# Autodesk Inventor assembly: Flash_Hobby_D3536EVO
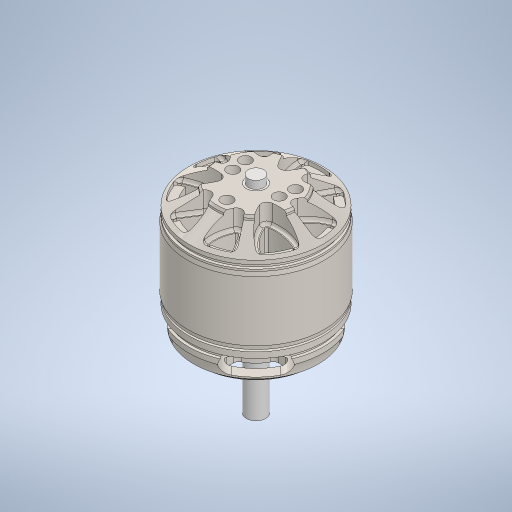
[picture p0: Inventor's stored thumbnail of the model, 512x512]
Saved by Autodesk Inventor 2023.2 (Build 272271000, 271)
## iProperties
Created: 2023-05-23
Part Number: Flash_Hobby_D3536EVO
Document SubType Name: Assembly
Designer: Nathan Cai
Mass: 105.8 g
Surface Area: 143.212 cm^2
Volume: 20.9807 cm^3
Sending System: Autodesk Translation Framework v12.4.0.73
Preprocessor: ST-DEVELOPER v19.2
Title: Flash_Hobby_D3536EVO v3.step
## Documents named in this file (4)
- E:\Documents\Inventor\Chort V2.0\Flash_Hobby_D3536EVO v3\Flash_Hobby_D3536EVO v3.iam
- E:\Documents\Inventor\Chort V2.0\Flash_Hobby_D3536EVO v3\Component1.ipt
- E:\Documents\Inventor\Chort V2.0\Flash_Hobby_D3536EVO v3\Part5.ipt
- E:\Documents\Inventor\Chort V2.0\Shaft.ipt
## Components (3 placed, 3 different names)
1. Component1:1
2. Part5 — Mate:1, Flush:1
3. Shaft:1 — Mate:1, Flush:1
## Relationships (2: Mate 1, Flush 1)
- Mate:1: Part5 ↔ Shaft:1
- Flush:1: Part5 ↔ Shaft:1
